# Autodesk Inventor assembly: EnsembleAvant
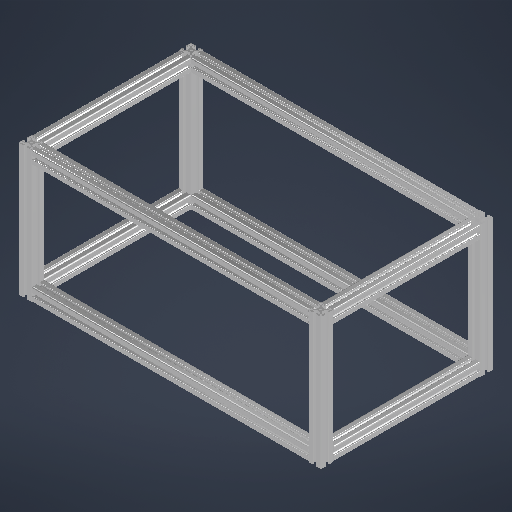
[picture p0: Inventor's stored thumbnail of the model, 512x512]
Saved by Autodesk Inventor 2026.2 (Build 302298010, 298A)
## iProperties
Part Number: EnsembleAvant
Document SubType Name: Ensemble
Designer: quent
Author: quent
## Documents named in this file (4)
- C:\Users\quent\OneDrive\Bureau\Master 2\Q2\Projet\EcoShell3D_VF\EnsembleAvant.iam
- C:\Users\quent\OneDrive\Bureau\Master 2\Q2\Projet\EcoShell3D_VF\profileAluAvant2.ipt
- C:\Users\quent\OneDrive\Bureau\Master 2\Q2\Projet\EcoShell3D_VF\profileAluAvant1.ipt
- C:\Users\quent\OneDrive\Bureau\Master 2\Q2\Projet\EcoShell3D_VF\profileAluAvant3.ipt
## Components (12 placed, 3 different names)
1. profileAluAvant2:1 — Placage:1, Affleurement:3, Affleurement:5, Placage:3, Affleurement:7, Affleurement:21, Affleurement:22, Placage:6, Affleurement:23
2. profileAluAvant2:2 — Placage:1, Affleurement:3, Placage:2, Affleurement:4, Affleurement:8, Affleurement:14, Affleurement:18, Placage:4, Affleurement:19, Affleurement:27, Affleurement:28
3. profileAluAvant2:3 — Placage:2, Affleurement:4, Affleurement:10, Affleurement:16, Placage:8, Placage:9
4. profileAluAvant2:4 — Affleurement:5, Placage:3, Affleurement:32, Affleurement:33, Placage:12
5. profileAluAvant1:1 — Affleurement:10, Affleurement:12, Affleurement:29, Placage:11
6. profileAluAvant1:2 — Affleurement:7, Affleurement:8, Affleurement:12, Affleurement:17, Placage:5, Affleurement:20
7. profileAluAvant1:3 — Affleurement:16, Affleurement:30, Affleurement:31, Placage:10
8. profileAluAvant1:4 — Affleurement:14, Affleurement:24, Affleurement:25, Placage:7, Affleurement:26
9. profileAluAvant3:1 — Affleurement:20, Affleurement:21, Affleurement:22, Placage:6, Placage:11, Placage:12
10. profileAluAvant3:2 — Affleurement:26, Affleurement:27, Affleurement:28, Placage:9, Affleurement:30, Affleurement:31
11. profileAluAvant3:3 — Affleurement:23, Affleurement:24, Affleurement:25, Placage:7, Placage:10, Affleurement:32, Affleurement:33
12. profileAluAvant3:4 — Affleurement:17, Affleurement:18, Placage:4, Placage:5, Affleurement:19, Affleurement:29, Placage:8
## Relationships (38: Flush 26, Mate 12)
- Placage:1 [Mate] (632 mm): profileAluAvant2:1 ↔ profileAluAvant2:2
- Affleurement:3 [Flush]: profileAluAvant2:1 ↔ profileAluAvant2:2
- Placage:2 [Mate] (241.624 mm): profileAluAvant2:2 ↔ profileAluAvant2:3
- Affleurement:4 [Flush]: profileAluAvant2:2 ↔ profileAluAvant2:3
- Affleurement:5 [Flush]: profileAluAvant2:1 ↔ profileAluAvant2:4
- Placage:3 [Mate] (241.624 mm): profileAluAvant2:1 ↔ profileAluAvant2:4
- Affleurement:7 [Flush]: profileAluAvant2:1 ↔ profileAluAvant1:2
- Affleurement:8 [Flush]: profileAluAvant2:2 ↔ profileAluAvant1:2
- Affleurement:10 [Flush]: profileAluAvant2:3 ↔ profileAluAvant1:1
- Affleurement:12 [Flush]: profileAluAvant1:1 ↔ profileAluAvant1:2
- Affleurement:14 [Flush]: profileAluAvant2:2 ↔ profileAluAvant1:4
- Affleurement:16 [Flush]: profileAluAvant2:3 ↔ profileAluAvant1:3
- Affleurement:17 [Flush]: profileAluAvant1:2 ↔ profileAluAvant3:4
- Affleurement:18 [Flush]: profileAluAvant2:2 ↔ profileAluAvant3:4
- Placage:4 [Mate]: profileAluAvant2:2 ↔ profileAluAvant3:4
- Placage:5 [Mate]: profileAluAvant1:2 ↔ profileAluAvant3:4
- Affleurement:19 [Flush]: profileAluAvant2:2 ↔ profileAluAvant3:4
- Affleurement:20 [Flush]: profileAluAvant1:2 ↔ profileAluAvant3:1
- Affleurement:21 [Flush]: profileAluAvant2:1 ↔ profileAluAvant3:1
- Affleurement:22 [Flush]: profileAluAvant2:1 ↔ profileAluAvant3:1
- Placage:6 [Mate]: profileAluAvant2:1 ↔ profileAluAvant3:1
- Affleurement:23 [Flush]: profileAluAvant2:1 ↔ profileAluAvant3:3
- Affleurement:24 [Flush]: profileAluAvant1:4 ↔ profileAluAvant3:3
- Affleurement:25 [Flush]: profileAluAvant1:4 ↔ profileAluAvant3:3
- Placage:7 [Mate]: profileAluAvant1:4 ↔ profileAluAvant3:3
- Affleurement:26 [Flush]: profileAluAvant1:4 ↔ profileAluAvant3:2
- Affleurement:27 [Flush]: profileAluAvant2:2 ↔ profileAluAvant3:2
- Affleurement:28 [Flush]: profileAluAvant2:2 ↔ profileAluAvant3:2
- Affleurement:29 [Flush]: profileAluAvant1:1 ↔ profileAluAvant3:4
- Placage:8 [Mate]: profileAluAvant2:3 ↔ profileAluAvant3:4
- Placage:9 [Mate]: profileAluAvant2:3 ↔ profileAluAvant3:2
- Affleurement:30 [Flush]: profileAluAvant1:3 ↔ profileAluAvant3:2
- Affleurement:31 [Flush]: profileAluAvant1:3 ↔ profileAluAvant3:2
- Placage:10 [Mate]: profileAluAvant1:3 ↔ profileAluAvant3:3
- Placage:11 [Mate]: profileAluAvant1:1 ↔ profileAluAvant3:1
- Affleurement:32 [Flush]: profileAluAvant2:4 ↔ profileAluAvant3:3
- Affleurement:33 [Flush]: profileAluAvant2:4 ↔ profileAluAvant3:3
- Placage:12 [Mate]: profileAluAvant2:4 ↔ profileAluAvant3:1
